# Autodesk Inventor assembly: RT_FRM_A_003_FrameV6
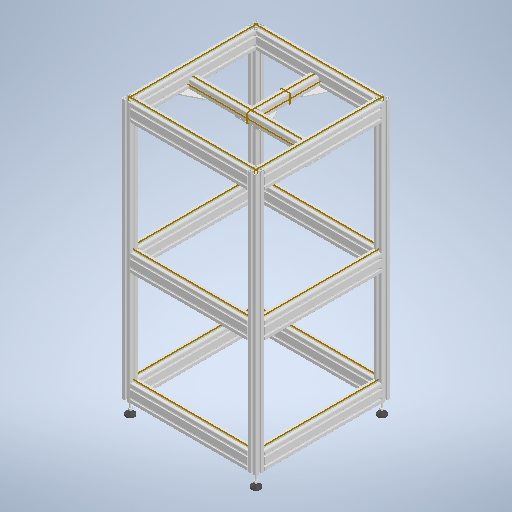
[picture p0: Inventor's stored thumbnail of the model, 512x512]
Saved by Autodesk Inventor 2025.3 (Build 293356000, 356)
## iProperties
Created: 2026-09-24
Part Number: RT_FRM_A_003_FrameV6
Document SubType Name: Assembly
Designer: louis
Author: louis
## Documents named in this file (7)
- C:\Dev\R_Trident\02_CAD\04_Subassemblies\RT_FRM_A_003_FrameV6.iam
- C:\Dev\R_Trident\02_CAD\01_Standard_Parts\02_FRM_FULL_Frame_V1\540_Profile_40x80L.ipt
- C:\Dev\R_Trident\02_CAD\01_Standard_Parts\02_FRM_FULL_Frame_V1\1200_Profile_40L.ipt
- C:\Dev\R_Trident\02_CAD\01_Standard_Parts\02_FRM_FULL_Frame_V1\BD40-8x50.ipt
- C:\Dev\R_Trident\02_CAD\01_Standard_Parts\02_FRM_FULL_Frame_V1\540_Profile_40L.ipt
- C:\Dev\R_Trident\02_CAD\01_Standard_Parts\02_FRM_FULL_Frame_V1\270_Profile_40L.ipt
- C:\Dev\R_Trident\02_CAD\01_Standard_Parts\02_FRM_FULL_Frame_V1\Motedis_LP40111.ipt
## Components (26 placed, 6 different names)
1. 1200_Profile_40L:1 — Mate:1, Flush:1, Flush:2, Mate:3, Flush:5, Flush:6, Mate:11, Mate:14, Flush:29, Mate:20, Mate:25
2. 1200_Profile_40L:2 — Flush:3, Flush:4, Mate:2, Mate:4, Flush:7, Flush:8, Flush:22, Flush:23, Mate:13, Mate:15, Mate:21
3. 1200_Profile_40L:3 — Mate:5, Flush:9, Flush:10, Flush:18, Mate:10, Flush:20, Flush:21, Mate:12, Flush:30, Mate:22
4. 1200_Profile_40L:4 — Flush:11, Flush:12, Mate:6, Flush:13, Mate:7, Flush:14, Flush:15, Mate:8, Flush:16, Flush:17, Flush:19, Mate:9, Flush:27, Flush:28, Mate:19, Mate:26
5. 540_Profile_40x80L:1 — Mate:1, Flush:1, Flush:2, Flush:13, Mate:7, Flush:14, Flush:15, Symmetry:2, Flush:32, Mate:39, Mate:42
6. 540_Profile_40x80L:2 — Flush:22, Flush:23, Mate:11, Symmetry:1, Symmetry:3, Mate:16, Mate:24
7. 540_Profile_40x80L:3 — Flush:3, Flush:4, Mate:2, Mate:28, Mate:46, Mate:48
8. 540_Profile_40x80L:4 — Mate:3, Flush:5, Flush:6, Mate:4, Flush:7, Flush:8, Mate:29, Mate:33
9. 540_Profile_40x80L:5 — Mate:5, Flush:9, Flush:10, Flush:11, Flush:12, Mate:6, Symmetry:1, Symmetry:3
10. 540_Profile_40x80L:6 — Mate:8, Flush:16, Flush:17
11. 540_Profile_40x80L:7 — Flush:18, Flush:19, Mate:9, Mate:23
12. 540_Profile_40x80L:8 — Mate:15, Flush:24, Flush:26, Flush:27
13. 540_Profile_40x80L:9 — Mate:13, Flush:25, Flush:30
14. 540_Profile_40x80L:10 — Mate:10, Flush:20, Flush:21, Symmetry:2
15. 540_Profile_40x80L:11 — Mate:12, Flush:24, Flush:25, Flush:29
16. 540_Profile_40x80L:12 — Mate:14, Flush:26, Flush:28
17. BD40-8x50:1 — Mate:19, Mate:26
18. BD40-8x50:2 — Mate:20, Mate:25
19. BD40-8x50:3 — Mate:21, Mate:24
20. BD40-8x50:4 — Mate:22, Mate:23
21. 540_Profile_40L:1 — Mate:27, Flush:31, Flush:32, Mate:28, Mate:34, Mate:35, Mate:37, Mate:38, Mate:40, Mate:41, Mate:44, Mate:45, Mate:47
22. 270_Profile_40L:1 — Mate:27, Flush:31, Mate:29, Mate:30, Mate:31, Mate:32, Mate:34, Mate:36, Mate:43
23. Motedis_LP40111:1 — Mate:44, Mate:45, Mate:46, Mate:47, Mate:48
24. Motedis_LP40111:2 — Mate:30, Mate:31, Mate:32, Mate:33
25. Motedis_LP40111:3 — Mate:38, Mate:39, Mate:40, Mate:41, Mate:42
26. Motedis_LP40111:4 — Mate:35, Mate:36, Mate:37, Mate:43
## Relationships (83: Mate 48, Flush 32, Symmetry 3)
- Mate:1: 1200_Profile_40L:1 ↔ 540_Profile_40x80L:1
- Flush:1: 1200_Profile_40L:1 ↔ 540_Profile_40x80L:1
- Flush:2: 1200_Profile_40L:1 ↔ 540_Profile_40x80L:1
- Flush:3: 1200_Profile_40L:2 ↔ 540_Profile_40x80L:3
- Flush:4: 1200_Profile_40L:2 ↔ 540_Profile_40x80L:3
- Mate:2: 1200_Profile_40L:2 ↔ 540_Profile_40x80L:3
- Mate:3: 1200_Profile_40L:1 ↔ 540_Profile_40x80L:4
- Flush:5: 1200_Profile_40L:1 ↔ 540_Profile_40x80L:4
- Flush:6: 1200_Profile_40L:1 ↔ 540_Profile_40x80L:4
- Mate:4: 1200_Profile_40L:2 ↔ 540_Profile_40x80L:4
- Flush:7: 1200_Profile_40L:2 ↔ 540_Profile_40x80L:4
- Flush:8: 1200_Profile_40L:2 ↔ 540_Profile_40x80L:4
- Mate:5: 1200_Profile_40L:3 ↔ 540_Profile_40x80L:5
- Flush:9: 1200_Profile_40L:3 ↔ 540_Profile_40x80L:5
- Flush:10: 1200_Profile_40L:3 ↔ 540_Profile_40x80L:5
- Flush:11: 1200_Profile_40L:4 ↔ 540_Profile_40x80L:5
- Flush:12: 1200_Profile_40L:4 ↔ 540_Profile_40x80L:5
- Mate:6: 1200_Profile_40L:4 ↔ 540_Profile_40x80L:5
- Flush:13: 1200_Profile_40L:4 ↔ 540_Profile_40x80L:1
- Mate:7: 1200_Profile_40L:4 ↔ 540_Profile_40x80L:1
- Flush:14: 1200_Profile_40L:4 ↔ 540_Profile_40x80L:1
- Flush:15: 1200_Profile_40L:4 ↔ 540_Profile_40x80L:1
- Mate:8: 1200_Profile_40L:4 ↔ 540_Profile_40x80L:6
- Flush:16: 1200_Profile_40L:4 ↔ 540_Profile_40x80L:6
- Flush:17: 1200_Profile_40L:4 ↔ 540_Profile_40x80L:6
- Flush:18: 1200_Profile_40L:3 ↔ 540_Profile_40x80L:7
- Flush:19: 1200_Profile_40L:4 ↔ 540_Profile_40x80L:7
- Mate:9: 1200_Profile_40L:4 ↔ 540_Profile_40x80L:7
- Mate:10: 1200_Profile_40L:3 ↔ 540_Profile_40x80L:10
- Flush:20: 1200_Profile_40L:3 ↔ 540_Profile_40x80L:10
- Flush:21: 1200_Profile_40L:3 ↔ 540_Profile_40x80L:10
- Flush:22: 1200_Profile_40L:2 ↔ 540_Profile_40x80L:2
- Flush:23: 1200_Profile_40L:2 ↔ 540_Profile_40x80L:2
- Mate:11: 1200_Profile_40L:1 ↔ 540_Profile_40x80L:2
- Mate:12: 1200_Profile_40L:3 ↔ 540_Profile_40x80L:11
- Mate:13: 1200_Profile_40L:2 ↔ 540_Profile_40x80L:9
- Mate:14: 1200_Profile_40L:1 ↔ 540_Profile_40x80L:12
- Mate:15: 1200_Profile_40L:2 ↔ 540_Profile_40x80L:8
- Flush:24: 540_Profile_40x80L:8 ↔ 540_Profile_40x80L:11
- Flush:25: 540_Profile_40x80L:9 ↔ 540_Profile_40x80L:11
- Flush:26: 540_Profile_40x80L:8 ↔ 540_Profile_40x80L:12
- Flush:27: 1200_Profile_40L:4 ↔ 540_Profile_40x80L:8
- Flush:28: 1200_Profile_40L:4 ↔ 540_Profile_40x80L:12
- Flush:29: 1200_Profile_40L:1 ↔ 540_Profile_40x80L:11
- Flush:30: 1200_Profile_40L:3 ↔ 540_Profile_40x80L:9
- Symmetry:1: 540_Profile_40x80L:2 ↔ 540_Profile_40x80L:5
- Symmetry:2: 540_Profile_40x80L:1 ↔ 540_Profile_40x80L:10
- Symmetry:3: 540_Profile_40x80L:2 ↔ 540_Profile_40x80L:5
- Mate:16: 540_Profile_40x80L:2
- Mate:17
- Mate:18
- Mate:19: 1200_Profile_40L:4 ↔ BD40-8x50:1
- Mate:20: 1200_Profile_40L:1 ↔ BD40-8x50:2
- Mate:21: 1200_Profile_40L:2 ↔ BD40-8x50:3
- Mate:22: 1200_Profile_40L:3 ↔ BD40-8x50:4
- Mate:23: 540_Profile_40x80L:7 ↔ BD40-8x50:4
- Mate:24: 540_Profile_40x80L:2 ↔ BD40-8x50:3
- Mate:25: 1200_Profile_40L:1 ↔ BD40-8x50:2
- Mate:26: 1200_Profile_40L:4 ↔ BD40-8x50:1
- Mate:27: 540_Profile_40L:1 ↔ 270_Profile_40L:1
- Flush:31: 540_Profile_40L:1 ↔ 270_Profile_40L:1
- Flush:32: 540_Profile_40x80L:1 ↔ 540_Profile_40L:1
- Mate:28: 540_Profile_40x80L:3 ↔ 540_Profile_40L:1
- Mate:29: 540_Profile_40x80L:4 ↔ 270_Profile_40L:1
- Mate:30: 270_Profile_40L:1 ↔ Motedis_LP40111:2
- Mate:31: 270_Profile_40L:1 ↔ Motedis_LP40111:2
- Mate:32: 270_Profile_40L:1 ↔ Motedis_LP40111:2
- Mate:33: 540_Profile_40x80L:4 ↔ Motedis_LP40111:2
- Mate:34: 540_Profile_40L:1 ↔ 270_Profile_40L:1
- Mate:35: 540_Profile_40L:1 ↔ Motedis_LP40111:4
- Mate:36: 270_Profile_40L:1 ↔ Motedis_LP40111:4
- Mate:37: 540_Profile_40L:1 ↔ Motedis_LP40111:4
- Mate:38: 540_Profile_40L:1 ↔ Motedis_LP40111:3
- Mate:39: 540_Profile_40x80L:1 ↔ Motedis_LP40111:3
- Mate:40: 540_Profile_40L:1 ↔ Motedis_LP40111:3
- Mate:41: 540_Profile_40L:1 ↔ Motedis_LP40111:3
- Mate:42: 540_Profile_40x80L:1 ↔ Motedis_LP40111:3
- Mate:43: 270_Profile_40L:1 ↔ Motedis_LP40111:4
- Mate:44: 540_Profile_40L:1 ↔ Motedis_LP40111:1
- Mate:45: 540_Profile_40L:1 ↔ Motedis_LP40111:1
- Mate:46: 540_Profile_40x80L:3 ↔ Motedis_LP40111:1
- Mate:47: 540_Profile_40L:1 ↔ Motedis_LP40111:1
- Mate:48: 540_Profile_40x80L:3 ↔ Motedis_LP40111:1
